# Autodesk Inventor assembly: assembly_completo
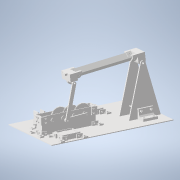
[picture p0: Inventor's stored thumbnail of the model, 180x180]
Saved by Autodesk Inventor 2022 (Build 260153000, 153)
## iProperties
Created: 2022-03-18
Part Number: assembly_completo
Document SubType Name: Assembly
Designer: jrdia
Author: jrdia
## Documents named in this file (16)
- D:\Semestre_9\Diseño_Innovación_1\mini1_diseno\archivos_stl\assembly_completo.iam
- D:\Semestre_9\Diseño_Innovación_1\mini1_diseno\base.ipt
- D:\Semestre_9\Diseño_Innovación_1\mini1_diseno\bisagra_base.ipt
- D:\Semestre_9\Diseño_Innovación_1\mini1_diseno\pared.ipt
- D:\Semestre_9\Diseño_Innovación_1\mini1_diseno\union_superior.ipt
- D:\Semestre_9\Diseño_Innovación_1\mini1_diseno\carril.ipt
- D:\Semestre_9\Diseño_Innovación_1\mini1_diseno\union_extremoV2.ipt
- D:\Semestre_9\Diseño_Innovación_1\mini1_diseno\Assembly1.iam
- D:\Semestre_9\Diseño_Innovación_1\mini1_diseno\escuadra_motor.ipt
- D:\Semestre_9\Diseño_Innovación_1\mini1_diseno\pared_motor.ipt
- D:\Semestre_9\Diseño_Innovación_1\mini1_diseno\base_motor.ipt
- D:\Semestre_9\Diseño_Innovación_1\mini1_diseno\acople.ipt
- D:\Semestre_9\Diseño_Innovación_1\mini1_diseno\eslabon_grande.ipt
- D:\Semestre_9\Diseño_Innovación_1\mini1_diseno\eslabon_pequeno.ipt
- D:\Semestre_9\Diseño_Innovación_1\mini1_diseno\archivos_stl\Assembly_cajaplaca.iam
- D:\Semestre_9\Diseño_Innovación_1\mini1_diseno\archivos_stl\Assembly_cajativa.iam
## Components (21 placed, 15 different names)
1. base:1 — Rotational:1, Mate:1, Rotational:2, Mate:2, Rotational:10, Mate:5, Rotational:15, Mate:6, Rotational:17, Rotational:18, Rotational:19
2. bisagra_base:1 — Rotational:1, Mate:1, Rotational:3, Mate:3
3. bisagra_base:2 — Rotational:2, Mate:2, Rotational:4, Mate:4
4. pared:1 — Rotational:3, Mate:3, Rotational:5
5. pared:2 — Rotational:4, Mate:4
6. union_superior:1 — Rotational:5, Rotational:6, Rotational:8
7. carril:1 — Rotational:6, Rotational:7
8. carril:2 — Rotational:8, Rotational:9
9. union_extremoV2:1 — Rotational:7, Rotational:9, Mate:13
10. Assembly1:1 [sub-assembly] — Rotational:10, Mate:5, Mate:7, Mate:8, Mate:9, Mate:10, Mate:11, Mate:12
11. escuadra_motor:1 — Rotational:13, Rotational:15
12. escuadra_motor:2 — Rotational:14, Mate:6
13. pared_motor:1 — Rotational:11, Rotational:14
14. pared_motor:2 — Rotational:12, Rotational:13
15. base_motor:1 — Rotational:11, Rotational:12
16. acople:1 — Mate:7, Mate:8, Mate:9
17. eslabon_grande:1 — Rotational:16, Mate:13
18. eslabon_pequeno:1 — Mate:10, Mate:11, Mate:12, Rotational:16
19. Assembly_cajaplaca:1 [sub-assembly] — Rotational:17
20. Assembly_cajaplaca:2 [sub-assembly] — Rotational:18
21. Assembly_cajativa:1 [sub-assembly] — Rotational:19
## Relationships (32: RevoluteJoint 19, Mate 13)
- Rotational:1 [RevoluteJoint]: base:1 ↔ bisagra_base:1
- Mate:1: base:1 ↔ bisagra_base:1
- Rotational:2 [RevoluteJoint]: base:1 ↔ bisagra_base:2
- Mate:2: base:1 ↔ bisagra_base:2
- Rotational:3 [RevoluteJoint]: bisagra_base:1 ↔ pared:1
- Mate:3: bisagra_base:1 ↔ pared:1
- Rotational:4 [RevoluteJoint]: bisagra_base:2 ↔ pared:2
- Mate:4: bisagra_base:2 ↔ pared:2
- Rotational:5 [RevoluteJoint]: pared:1 ↔ union_superior:1
- Rotational:6 [RevoluteJoint]: union_superior:1 ↔ carril:1
- Rotational:7 [RevoluteJoint]: carril:1 ↔ union_extremoV2:1
- Rotational:8 [RevoluteJoint]: union_superior:1 ↔ carril:2
- Rotational:9 [RevoluteJoint]: carril:2 ↔ union_extremoV2:1
- Rotational:10 [RevoluteJoint]: base:1 ↔ Assembly1:1
- Mate:5: base:1 ↔ Assembly1:1
- Rotational:11 [RevoluteJoint]: pared_motor:1 ↔ base_motor:1
- Rotational:12 [RevoluteJoint]: pared_motor:2 ↔ base_motor:1
- Rotational:13 [RevoluteJoint]: escuadra_motor:1 ↔ pared_motor:2
- Rotational:14 [RevoluteJoint]: escuadra_motor:2 ↔ pared_motor:1
- Rotational:15 [RevoluteJoint]: base:1 ↔ escuadra_motor:1
- Mate:6: base:1 ↔ escuadra_motor:2
- Mate:7: Assembly1:1 ↔ acople:1
- Mate:8: Assembly1:1 ↔ acople:1
- Mate:9 (5 mm): Assembly1:1 ↔ acople:1
- Mate:10 (10 mm): Assembly1:1 ↔ eslabon_pequeno:1
- Mate:11: Assembly1:1 ↔ eslabon_pequeno:1
- Mate:12: Assembly1:1 ↔ eslabon_pequeno:1
- Rotational:16 [RevoluteJoint]: eslabon_grande:1 ↔ eslabon_pequeno:1
- Mate:13: union_extremoV2:1 ↔ eslabon_grande:1
- Rotational:17 [RevoluteJoint]: base:1 ↔ Assembly_cajaplaca:1
- Rotational:18 [RevoluteJoint]: base:1 ↔ Assembly_cajaplaca:2
- Rotational:19 [RevoluteJoint]: base:1 ↔ Assembly_cajativa:1
